# Autodesk Inventor assembly: fork
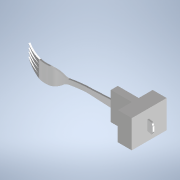
[picture p0: Inventor's stored thumbnail of the model, 180x180]
Saved by Autodesk Inventor 2022 (Build 260153000, 153)
## iProperties
Created: 2022-10-23
Part Number: fork
Document SubType Name: Assembly
Designer: Yazawa
Author: Yazawa
## Documents named in this file (3)
- C:\Users\Yazawa\Documents\GitHub\fork\fork.iam
- C:\Users\Yazawa\Documents\GitHub\fork\fork.ipt
- C:\Users\Yazawa\Documents\GitHub\fork\forkmount.ipt
## Components (2 placed, 2 different names)
1. fork:1 — フラッシュ:1
2. forkmount:1 — フラッシュ:1
## Relationships (1: Flush 1)
- フラッシュ:1 [Flush]: fork:1 ↔ forkmount:1
